# Autodesk Inventor assembly: duplex
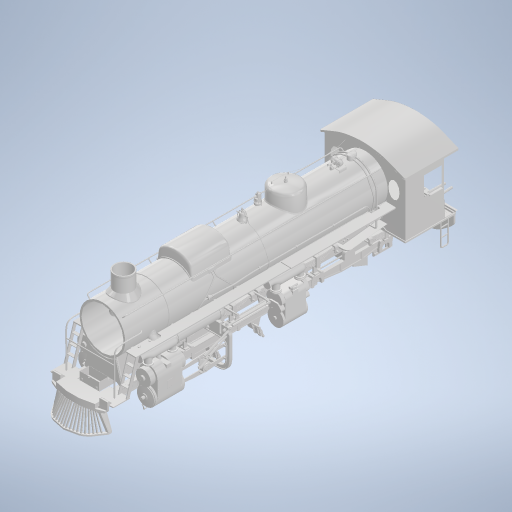
[picture p0: Inventor's stored thumbnail of the model, 512x512]
Saved by Autodesk Inventor 2023 (Build 270158000, 158)
## iProperties
Created: 2023-09-11
Part Number: duplex
Document SubType Name: Assembly
Designer: Peter
Author: Peter
## Documents named in this file (16)
- D:\code\dv-rearranged-S282\models\duplex.iam
- D:\code\dv-rearranged-S282\models\dry_pipe.ipt
- D:\code\dv-rearranged-S282\models\s282_mesh.ipt
- D:\code\dv-rearranged-S282\models\cylinder.ipt
- D:\code\dv-rearranged-S282\models\dry_pipe_left.ipt
- D:\code\dv-rearranged-S282\models\intake_manifold_r.ipt
- D:\code\dv-rearranged-S282\models\intake_manifold_f.ipt
- D:\code\dv-rearranged-S282\models\dry_pipe_new.ipt
- D:\code\dv-rearranged-S282\models\transmission_box.ipt
- D:\code\dv-rearranged-S282\models\u_joint.ipt
- D:\code\dv-rearranged-S282\models\driveshaft_r.ipt
- D:\code\dv-rearranged-S282\models\transmission_box_mount_shaft.ipt
- D:\code\dv-rearranged-S282\models\driveshaft_f.ipt
- D:\code\dv-rearranged-S282\models\driveshaft_m.ipt
- D:\code\dv-rearranged-S282\models\driveshaft_m_mount_shaft.ipt
- D:\code\dv-rearranged-S282\models\mount_shaft_mount.ipt
## Components (19 placed, 17 different names)
1. dry_pipe:1
2. s282_mesh:1
3. cylinderLR — Mate:2, Mate:3
4. dry_pipe_left:1
5. cylinderRR
6. intake_manifold_LR — Mate:2, Mate:3
7. intake_manifold_RR
8. intake_manifold_f:1
9. dry_pipe_new:1
10. intake_manifold_f:2
11. transmission_box:1 — Flush:1
12. u_joint:1 — Flush:1
13. u_joint:2 — Flush:2, Mate:4
14. driveshaft_r:1 — Flush:2, Mate:4
15. transmission_box_mount_shaft:1
16. driveshaft_f:1
17. driveshaft_m:1
18. driveshaft_m_mount_shaft:1
19. mount_shaft_mount:1
## Relationships (5: Mate 3, Flush 2)
- Mate:2 (15.24 mm): cylinderLR ↔ intake_manifold_LR
- Mate:3: cylinderLR ↔ intake_manifold_LR
- Flush:1: transmission_box:1 ↔ u_joint:1
- Flush:2: u_joint:2 ↔ driveshaft_r:1
- Mate:4: u_joint:2 ↔ driveshaft_r:1
